# Autodesk Inventor assembly: rudder
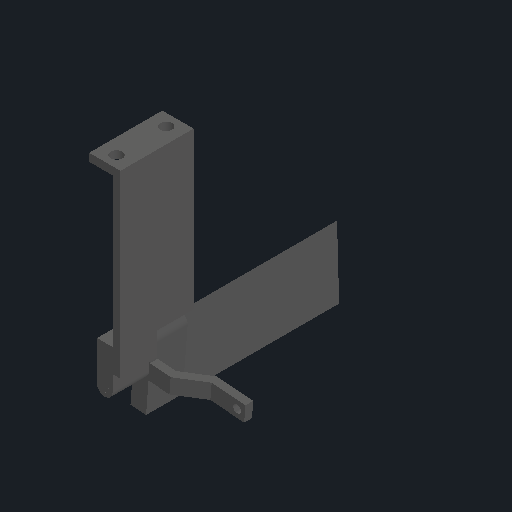
[picture p0: Inventor's stored thumbnail of the model, 512x512]
Saved by Autodesk Inventor 2022.2 (Build 262287010, 287A)
## iProperties
Created: 2022-03-30
Part Number: rudder
Document SubType Name: Assembly
Designer: kardo
Author: kardo
## Documents named in this file (3)
- D:\Computer Aided Design\hydroplane_plan_2_refactor\model\shape\frame\hardware\rudder.iam
- D:\Computer Aided Design\hydroplane_plan_2_refactor\model\shape\frame\hardware\rudder_base.ipt
- D:\Computer Aided Design\hydroplane_plan_2_refactor\model\shape\frame\hardware\rudder_fin.ipt
## Components (2 placed, 2 different names)
1. rudder_base:1 — Cylindrical:1
2. rudder_fin:1 — Cylindrical:1
## Relationships (1: CylindricalJoint 1)
- Cylindrical:1: rudder_base:1 ↔ rudder_fin:1
